# Autodesk Inventor assembly: End Ramp Assembly
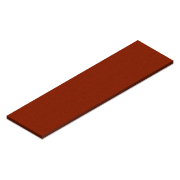
[picture p0: Inventor's stored thumbnail of the model, 180x180]
Saved by Autodesk Inventor 2015 (Build 190159000, 159)
## iProperties
Created: 2015-01-20
Part Number: End Ramp Assembly
Document SubType Name: Assembly
Designer: Peter
Author: Peter
## Documents named in this file (3)
- T:\FILES\FIRST-Team-1719-CAD-Team\2015 Playing Field\Team 1719 Practice Field\Scoring Platform - Construction Design\End Ramp Assembly.iam
- T:\FILES\FIRST-Team-1719-CAD-Team\2015 Playing Field\Team 1719 Practice Field\Scoring Platform - Construction Design\End Plywood Ramp 375.ipt
- T:\FILES\FIRST-Team-1719-CAD-Team\2015 Playing Field\Team 1719 Practice Field\Scoring Platform - Construction Design\End Clear Ramp Surface 125 - Version 2.ipt
## Components (2 placed, 2 different names)
1. End Plywood Ramp 375:1 — Mate:2, Flush:3
2. End Clear Ramp Surface 125 - Version 2:1 — Mate:2, Flush:3
## Relationships (2: Mate 1, Flush 1)
- Mate:2: End Plywood Ramp 375:1 ↔ End Clear Ramp Surface 125 - Version 2:1
- Flush:3: End Plywood Ramp 375:1 ↔ End Clear Ramp Surface 125 - Version 2:1
